# Autodesk Inventor assembly: Main Body
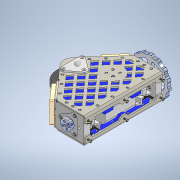
[picture p0: Inventor's stored thumbnail of the model, 180x180]
Saved by Autodesk Inventor 2022 (Build 260153000, 153)
## iProperties
Created: 2022-08-09
Part Number: Main Body
Document SubType Name: Assembly
Designer: Nick
Mass: 1334.27 g
Surface Area: 2820.47 cm^2
Volume: 520.306 cm^3
Density: 2.56439 g/cm^3
Author: Nick
## Documents named in this file (31)
- Y:\Projects\BattleBot\Main Body.iam
- Y:\Projects\BattleBot\Battery.ipt
- Y:\Projects\BattleBot\ESC.ipt
- Y:\Projects\BattleBot\Motor.ipt
- Y:\Projects\BattleBot\RC Reciever.ipt
- Y:\Projects\BattleBot\Base Plate.ipt
- Y:\Projects\BattleBot\Weapon.ipt
- Y:\Projects\BattleBot\Brushless Motor.ipt
- Y:\Projects\BattleBot\Brushed ESC.ipt
- Y:\Projects\BattleBot\Bottom Substructure.ipt
- Y:\Projects\BattleBot\Wheel.ipt
- Y:\Projects\BattleBot\6901 Bearing.ipt
- Y:\Projects\BattleBot\GT2 Pulley 16T.ipt
- Y:\Projects\BattleBot\Motor Mount Insert.ipt
- Y:\Projects\BattleBot\Mount Side.ipt
- Y:\Projects\BattleBot\Top Stubstructure.ipt
- Y:\Projects\BattleBot\Shaft.ipt
- Y:\Projects\BattleBot\Key.ipt
- Y:\Projects\BattleBot\ESC Mount.ipt
- Y:\Projects\BattleBot\Shaft Collar.ipt
- Y:\Projects\BattleBot\Wheel Hub.ipt
- Y:\Projects\BattleBot\Front Armor.ipt
- Y:\Projects\BattleBot\Rear Armor.ipt
- Y:\Projects\BattleBot\M3 Heat Set Insert.ipt
- Y:\Projects\BattleBot\M3 x 8 mm FHCS.ipt
- Y:\Projects\Mini_Sand_Table\Hardware\M3\Bolts\M3 x 8 mm FHCS.ipt
- Y:\Projects\BattleBot\M3 x 12 mm FHCS.ipt
- Y:\Projects\BattleBot\Motor Clamp.ipt
- Y:\Projects\BattleBot\Pulley.ipt
- Y:\Projects\BattleBot\Idle Ball Mount.ipt
- Y:\Projects\BattleBot\Ball.ipt
## Components (183 placed, 29 different names)
1. Battery:1 — Mate:146, Mate:182, Mate:189, Flush:39
2. ESC:1 — Mate:168, Mate:189, Flush:39, Mate:191
3. Base Plate:1 — Mate:42, Mate:95, Insert:15, Mate:104, Mate:105, Mate:139, Flush:28, Mate:140, Flush:29, Insert:123, Insert:124, Insert:125, Insert:126, Insert:127, Insert:128, Insert:129, Insert:130, Insert:131, Insert:132, Insert:133, Insert:134, Insert:135, Insert:136, Insert:137, Insert:138, Insert:183, Insert:184, Insert:185, Insert:189, Insert:190
4. Weapon:1 — Mate:145, Mate:159, Insert:33, Angle:1, Mate:187
5. Brushless Motor:1 — Insert:26, Insert:32
6. Motor:2 — Insert:22, Insert:36, Angle:2
7. Motor:3 — Insert:21, Insert:39, Angle:3
8. Brushed ESC:1 — Mate:128, Mate:132, Flush:37
9. Brushed ESC:2 — Mate:150, Mate:161
10. Bottom Substructure:2 — Mate:42, Mate:95, Mate:128, Mate:144, Flush:32, Mate:146, Mate:161, Mate:162, Mate:165, Mate:182, Insert:42, Insert:43, Insert:44, Insert:45, Insert:46, Insert:47, Insert:48, Insert:51, Insert:52, Insert:53, Insert:56, Insert:57, Insert:99, Insert:100, Insert:105, Insert:106, Mate:190
11. Base Plate:2 — Mate:125, Insert:32, Mate:173, Mate:174, Mate:178, Mate:179, Insert:107, Insert:108, Insert:109, Insert:110, Insert:111, Insert:112, Insert:113, Insert:114, Insert:115, Insert:116, Insert:117, Insert:118, Insert:119, Insert:120, Insert:121, Insert:122, Insert:139, Insert:140, Insert:141, Insert:142, Mate:183, Mate:185, Insert:186, Insert:187, Insert:188, Insert:192, Insert:193
12. Wheel:1 — Insert:34, Insert:195
13. Wheel:2 — Insert:37
14. 6901 Bearing:1 — Insert:15, Insert:27
15. GT2 Pulley 16T:1 — Insert:26
16. Motor Mount Insert:1 — Insert:22, Insert:30, Insert:31, Insert:147, Insert:148, Insert:149
17. Mount Side:1 — Mate:104, Mate:140, Flush:29, Mate:144, Mate:150, Mate:164, Mate:166, Insert:30, Insert:31, Flush:38, Insert:86, Insert:87, Insert:88, Insert:89, Insert:90, Insert:91, Insert:92, Insert:93, Insert:94, Insert:95, Insert:96, Insert:98
18. Mount Side:2 — Mate:105, Mate:132, Mate:139, Flush:28, Flush:30, Mate:141, Mate:163, Flush:36, Insert:28, Insert:29, Mate:180, Insert:72, Insert:73, Insert:74, Insert:75, Insert:76, Insert:77, Insert:78, Insert:79, Insert:81, Insert:82, Insert:83, Insert:84
19. Motor Mount Insert:3 — Insert:21, Insert:28, Insert:29, Insert:150, Insert:151, Insert:152
20. 6901 Bearing:2 — Insert:25
21. Top Stubstructure:1 — Mate:125, Insert:25, Flush:30, Mate:141, Insert:58, Insert:59, Insert:60, Insert:61, Insert:62, Insert:63, Insert:64, Insert:65, Insert:66, Insert:67, Insert:68, Insert:69, Insert:70, Insert:71, Insert:101, Insert:102, Insert:103, Insert:104
22. Shaft:1 — Insert:27, Mate:157, Mate:158, Mate:159, Mate:186
23. Key:1 — Mate:157, Mate:158, Angle:1, Angle:4
24. ESC Mount:1 — Mate:162, Mate:163, Flush:36, Flush:37, Insert:173, Insert:174, Insert:180, Angle:3
25. ESC Mount:2 — Mate:164, Mate:165, Mate:166, Mate:168, Insert:171, Insert:172, Insert:175, Insert:176, Angle:2
26. Shaft Collar:1 — Insert:33
27. Wheel Hub:1 — Insert:34, Insert:36, Insert:195
28. Wheel Hub:2 — Insert:37, Insert:39
29. Front Armor:1 — Mate:173, Flush:38, Mate:174, Mate:184, Insert:163, Insert:164, Insert:165, Insert:166
30. Front Armor:2 — Mate:183, Mate:184, Mate:185, Insert:167, Insert:168, Insert:169, Insert:170
31. Rear Armor:1 — Mate:178, Mate:179, Mate:180
32. Motor Clamp:1 — Insert:175, Insert:176, Insert:177, Insert:178
33. Motor Clamp:2 — Insert:179, Insert:180, Insert:181, Insert:182
34. Pulley:1 — Mate:186, Angle:4, Mate:187
35. Idle Ball Mount:1 — Insert:189, Insert:190, Insert:191
36. Idle Ball Mount:2 — Insert:192, Insert:193, Insert:194
37. Ball:1 — Insert:191
38. Ball:2 — Insert:194
39. RC Reciever:1 — Mate:190, Mate:191
40. M3 Heat Set Insert:67 — Insert:171
41. M3 Heat Set Insert:68 — Insert:172
42. M3 Heat Set Insert:69 — Insert:174
43. M3 Heat Set Insert:70 — Insert:173, Insert:179
44. M3 Heat Set Insert:1 — Insert:48
45. M3 Heat Set Insert:2 — Insert:47
46. M3 Heat Set Insert:3 — Insert:46
47. M3 Heat Set Insert:4 — Insert:45
48. M3 Heat Set Insert:5
49. M3 Heat Set Insert:6 — Insert:42
50. M3 Heat Set Insert:7 — Insert:43
51. M3 Heat Set Insert:8 — Insert:44
52. M3 Heat Set Insert:9
53. M3 Heat Set Insert:10 — Insert:51
54. M3 Heat Set Insert:11 — Insert:52
55. M3 Heat Set Insert:12 — Insert:53
56. M3 Heat Set Insert:13 — Insert:56
57. M3 Heat Set Insert:14
58. M3 Heat Set Insert:15
59. M3 Heat Set Insert:16
60. M3 Heat Set Insert:17
61. M3 Heat Set Insert:18 — Insert:57
62. M3 Heat Set Insert:19 — Insert:58
63. M3 Heat Set Insert:20 — Insert:59
64. M3 Heat Set Insert:21 — Insert:60
65. M3 Heat Set Insert:22 — Insert:61
66. M3 Heat Set Insert:23 — Insert:67
67. M3 Heat Set Insert:24 — Insert:66
68. M3 Heat Set Insert:25 — Insert:65
69. M3 Heat Set Insert:26 — Insert:64
70. M3 Heat Set Insert:27 — Insert:68
71. M3 Heat Set Insert:28 — Insert:69
72. M3 Heat Set Insert:29 — Insert:70
73. M3 Heat Set Insert:30 — Insert:71
74. M3 Heat Set Insert:31 — Insert:63
75. M3 Heat Set Insert:32 — Insert:62
76. M3 Heat Set Insert:33 — Insert:77
77. M3 Heat Set Insert:34 — Insert:76
78. M3 Heat Set Insert:35 — Insert:75
79. M3 Heat Set Insert:36 — Insert:78
80. M3 Heat Set Insert:37 — Insert:73
81. M3 Heat Set Insert:38 — Insert:72
82. M3 Heat Set Insert:39 — Insert:79
83. M3 Heat Set Insert:40 — Insert:74
84. M3 Heat Set Insert:41
85. M3 Heat Set Insert:42 — Insert:82
86. M3 Heat Set Insert:43 — Insert:83
87. M3 Heat Set Insert:44 — Insert:81
88. M3 Heat Set Insert:45 — Insert:84
89. M3 Heat Set Insert:46 — Insert:92
90. M3 Heat Set Insert:47 — Insert:87
91. M3 Heat Set Insert:48 — Insert:86
92. M3 Heat Set Insert:49 — Insert:98
93. M3 Heat Set Insert:50 — Insert:95
94. M3 Heat Set Insert:51 — Insert:91
95. M3 Heat Set Insert:52 — Insert:96
96. M3 Heat Set Insert:53 — Insert:94
97. M3 Heat Set Insert:54 — Insert:88
98. M3 Heat Set Insert:55 — Insert:90
99. M3 Heat Set Insert:56 — Insert:89
100. M3 Heat Set Insert:57 — Insert:93
101. M3 Heat Set Insert:58
102. M3 Heat Set Insert:59 — Insert:99
103. M3 Heat Set Insert:60 — Insert:100
104. M3 Heat Set Insert:61 — Insert:102
105. M3 Heat Set Insert:62 — Insert:101
106. M3 Heat Set Insert:63 — Insert:103
107. M3 Heat Set Insert:64 — Insert:105
108. M3 Heat Set Insert:65 — Insert:104
109. M3 Heat Set Insert:66 — Insert:106
110. M3 x 8 mm FHCS:51 — Insert:183
111. M3 x 8 mm FHCS:52 — Insert:184
112. M3 x 8 mm FHCS:53 — Insert:185
113. M3 x 8 mm FHCS:54 — Insert:186
114. M3 x 8 mm FHCS:55 — Insert:188
115. M3 x 8 mm FHCS:56 — Insert:187
116. M3 x 8 mm FHCS:1 — Insert:107
117. M3 x 8 mm FHCS:2 — Insert:108
118. M3 x 8 mm FHCS:3 — Insert:110
119. M3 x 8 mm FHCS:4 — Insert:109
120. M3 x 8 mm FHCS:5 — Insert:111
121. M3 x 8 mm FHCS:6 — Insert:112
122. M3 x 8 mm FHCS:7 — Insert:113
123. M3 x 8 mm FHCS:8 — Insert:114
124. M3 x 8 mm FHCS:9 — Insert:115
125. M3 x 8 mm FHCS:10 — Insert:116
126. M3 x 8 mm FHCS:11 — Insert:118
127. M3 x 8 mm FHCS:12 — Insert:119
128. M3 x 8 mm FHCS:13 — Insert:117
129. M3 x 8 mm FHCS:14 — Insert:120
130. M3 x 8 mm FHCS:15 — Insert:123
131. M3 x 8 mm FHCS:16 — Insert:122
132. M3 x 8 mm FHCS:17 — Insert:121
133. M3 x 8 mm FHCS:18 — Insert:124
134. M3 x 8 mm FHCS:19 — Insert:125
135. M3 x 8 mm FHCS:20 — Insert:126
136. M3 x 8 mm FHCS:21 — Insert:127
137. M3 x 8 mm FHCS:22 — Insert:128
138. M3 x 8 mm FHCS:23 — Insert:129
139. M3 x 8 mm FHCS:24 — Insert:130
140. M3 x 8 mm FHCS:25 — Insert:131
141. M3 x 8 mm FHCS:26 — Insert:132
142. M3 x 8 mm FHCS:27 — Insert:133
143. M3 x 8 mm FHCS:28 — Insert:134
144. M3 x 8 mm FHCS:29 — Insert:138
145. M3 x 8 mm FHCS:30 — Insert:137
146. M3 x 8 mm FHCS:31 — Insert:136
147. M3 x 8 mm FHCS:32 — Insert:135
148. M3 x 8 mm FHCS:33 — Insert:139
149. M3 x 8 mm FHCS:34 — Insert:140
150. M3 x 8 mm FHCS:35 — Insert:142
151. M3 x 8 mm FHCS:36 — Insert:141
152. M3 x 8 mm FHCS:37 — Insert:147
153. M3 x 8 mm FHCS:38 — Insert:148
154. M3 x 8 mm FHCS:39
155. M3 x 8 mm FHCS:40 — Insert:149
156. M3 x 8 mm FHCS:41
157. M3 x 8 mm FHCS:42
158. M3 x 8 mm FHCS:43
159. M3 x 8 mm FHCS:44
160. M3 x 8 mm FHCS:45 — Insert:152
161. M3 x 8 mm FHCS:46
162. M3 x 8 mm FHCS:47
163. M3 x 8 mm FHCS:48 — Insert:150
164. M3 x 8 mm FHCS:49 — Insert:151
165. M3 x 8 mm FHCS:50
166. M3 x 12 mm FHCS:15 — Insert:177
167. M3 x 12 mm FHCS:16 — Insert:178
168. M3 x 12 mm FHCS:17 — Insert:182
169. M3 x 12 mm FHCS:18 — Insert:181
170. M3 x 12 mm FHCS:1
171. M3 x 12 mm FHCS:2
172. M3 x 12 mm FHCS:3
173. M3 x 12 mm FHCS:4
174. M3 x 12 mm FHCS:5
175. M3 x 12 mm FHCS:6
176. M3 x 12 mm FHCS:7 — Insert:168
177. M3 x 12 mm FHCS:8 — Insert:167
178. M3 x 12 mm FHCS:9 — Insert:169
179. M3 x 12 mm FHCS:10 — Insert:170
180. M3 x 12 mm FHCS:11 — Insert:164
181. M3 x 12 mm FHCS:12 — Insert:163
182. M3 x 12 mm FHCS:13 — Insert:165
183. M3 x 12 mm FHCS:14 — Insert:166
## Relationships (199: Insert 149, Mate 38, Flush 8, Angle 4)
- Mate:42: Base Plate:1 ↔ Bottom Substructure:2
- Mate:95: Base Plate:1 ↔ Bottom Substructure:2
- Insert:15: Base Plate:1 ↔ 6901 Bearing:1
- Mate:104: Base Plate:1 ↔ Mount Side:1
- Mate:105: Base Plate:1 ↔ Mount Side:2
- Insert:21: Motor:3 ↔ Motor Mount Insert:3
- Insert:22: Motor:2 ↔ Motor Mount Insert:1
- Mate:125: Base Plate:2 ↔ Top Stubstructure:1
- Insert:25: 6901 Bearing:2 ↔ Top Stubstructure:1
- Mate:128: Brushed ESC:1 ↔ Bottom Substructure:2
- Mate:132: Brushed ESC:1 ↔ Mount Side:2
- Mate:139: Base Plate:1 ↔ Mount Side:2
- Flush:28: Base Plate:1 ↔ Mount Side:2
- Mate:140: Base Plate:1 ↔ Mount Side:1
- Flush:29: Base Plate:1 ↔ Mount Side:1
- Flush:30: Mount Side:2 ↔ Top Stubstructure:1
- Mate:141: Mount Side:2 ↔ Top Stubstructure:1
- Mate:144: Bottom Substructure:2 ↔ Mount Side:1
- Flush:32 (15.5 mm): Bottom Substructure:2
- Mate:145: Weapon:1
- Mate:146: Battery:1 ↔ Bottom Substructure:2
- Mate:150: Brushed ESC:2 ↔ Mount Side:1
- Insert:26: Brushless Motor:1 ↔ GT2 Pulley 16T:1
- Insert:27: 6901 Bearing:1 ↔ Shaft:1
- Mate:157: Shaft:1 ↔ Key:1
- Mate:158: Shaft:1 ↔ Key:1
- Mate:159: Weapon:1 ↔ Shaft:1
- Mate:161: Brushed ESC:2 ↔ Bottom Substructure:2
- Mate:162: Bottom Substructure:2 ↔ ESC Mount:1
- Mate:163: Mount Side:2 ↔ ESC Mount:1
- Flush:36: Mount Side:2 ↔ ESC Mount:1
- Flush:37: Brushed ESC:1 ↔ ESC Mount:1
- Mate:164: Mount Side:1 ↔ ESC Mount:2
- Mate:165: Bottom Substructure:2 ↔ ESC Mount:2
- Mate:166: Mount Side:1 ↔ ESC Mount:2
- Mate:168 (1 mm): ESC:1 ↔ ESC Mount:2
- Insert:28: Mount Side:2 ↔ Motor Mount Insert:3
- Insert:29: Mount Side:2 ↔ Motor Mount Insert:3
- Insert:30: Motor Mount Insert:1 ↔ Mount Side:1
- Insert:31: Motor Mount Insert:1 ↔ Mount Side:1
- Insert:32: Brushless Motor:1 ↔ Base Plate:2
- Insert:33: Weapon:1 ↔ Shaft Collar:1
- Angle:1 (180 deg): Weapon:1 ↔ Key:1
- Insert:34: Wheel:1 ↔ Wheel Hub:1
- Insert:36: Motor:2 ↔ Wheel Hub:1
- Insert:37: Wheel:2 ↔ Wheel Hub:2
- Insert:39: Motor:3 ↔ Wheel Hub:2
- Mate:173: Base Plate:2 ↔ Front Armor:1
- Flush:38: Mount Side:1 ↔ Front Armor:1
- Mate:174: Base Plate:2 ↔ Front Armor:1
- Mate:178: Base Plate:2 ↔ Rear Armor:1
- Mate:179: Base Plate:2 ↔ Rear Armor:1
- Mate:180: Mount Side:2 ↔ Rear Armor:1
- Mate:182: Battery:1 ↔ Bottom Substructure:2
- Insert:42: Bottom Substructure:2 ↔ M3 Heat Set Insert:6
- Insert:43: Bottom Substructure:2 ↔ M3 Heat Set Insert:7
- Insert:44: Bottom Substructure:2 ↔ M3 Heat Set Insert:8
- Insert:45: Bottom Substructure:2 ↔ M3 Heat Set Insert:4
- Insert:46: Bottom Substructure:2 ↔ M3 Heat Set Insert:3
- Insert:47: Bottom Substructure:2 ↔ M3 Heat Set Insert:2
- Insert:48: Bottom Substructure:2 ↔ M3 Heat Set Insert:1
- Insert:51: Bottom Substructure:2 ↔ M3 Heat Set Insert:10
- Insert:52: Bottom Substructure:2 ↔ M3 Heat Set Insert:11
- Insert:53: Bottom Substructure:2 ↔ M3 Heat Set Insert:12
- Insert:56: Bottom Substructure:2 ↔ M3 Heat Set Insert:13
- Insert:57: Bottom Substructure:2 ↔ M3 Heat Set Insert:18
- Insert:58: Top Stubstructure:1 ↔ M3 Heat Set Insert:19
- Insert:59: Top Stubstructure:1 ↔ M3 Heat Set Insert:20
- Insert:60: Top Stubstructure:1 ↔ M3 Heat Set Insert:21
- Insert:61: Top Stubstructure:1 ↔ M3 Heat Set Insert:22
- Insert:62: Top Stubstructure:1 ↔ M3 Heat Set Insert:32
- Insert:63: Top Stubstructure:1 ↔ M3 Heat Set Insert:31
- Insert:64: Top Stubstructure:1 ↔ M3 Heat Set Insert:26
- Insert:65: Top Stubstructure:1 ↔ M3 Heat Set Insert:25
- Insert:66: Top Stubstructure:1 ↔ M3 Heat Set Insert:24
- Insert:67: Top Stubstructure:1 ↔ M3 Heat Set Insert:23
- Insert:68: Top Stubstructure:1 ↔ M3 Heat Set Insert:27
- Insert:69: Top Stubstructure:1 ↔ M3 Heat Set Insert:28
- Insert:70: Top Stubstructure:1 ↔ M3 Heat Set Insert:29
- Insert:71: Top Stubstructure:1 ↔ M3 Heat Set Insert:30
- Insert:72: Mount Side:2 ↔ M3 Heat Set Insert:38
- Insert:73: Mount Side:2 ↔ M3 Heat Set Insert:37
- Insert:74: Mount Side:2 ↔ M3 Heat Set Insert:40
- Insert:75: Mount Side:2 ↔ M3 Heat Set Insert:35
- Insert:76: Mount Side:2 ↔ M3 Heat Set Insert:34
- Insert:77: Mount Side:2 ↔ M3 Heat Set Insert:33
- Insert:78: Mount Side:2 ↔ M3 Heat Set Insert:36
- Insert:79: Mount Side:2 ↔ M3 Heat Set Insert:39
- Insert:81: Mount Side:2 ↔ M3 Heat Set Insert:44
- Insert:82: Mount Side:2 ↔ M3 Heat Set Insert:42
- Insert:83: Mount Side:2 ↔ M3 Heat Set Insert:43
- Insert:84: Mount Side:2 ↔ M3 Heat Set Insert:45
- Insert:86: Mount Side:1 ↔ M3 Heat Set Insert:48
- Insert:87: Mount Side:1 ↔ M3 Heat Set Insert:47
- Insert:88: Mount Side:1 ↔ M3 Heat Set Insert:54
- Insert:89: Mount Side:1 ↔ M3 Heat Set Insert:56
- Insert:90: Mount Side:1 ↔ M3 Heat Set Insert:55
- Insert:91: Mount Side:1 ↔ M3 Heat Set Insert:51
- Insert:92: Mount Side:1 ↔ M3 Heat Set Insert:46
- Insert:93: Mount Side:1 ↔ M3 Heat Set Insert:57
- Insert:94: Mount Side:1 ↔ M3 Heat Set Insert:53
- Insert:95: Mount Side:1 ↔ M3 Heat Set Insert:50
- Insert:96: Mount Side:1 ↔ M3 Heat Set Insert:52
- Insert:98: Mount Side:1 ↔ M3 Heat Set Insert:49
- Insert:99: Bottom Substructure:2 ↔ M3 Heat Set Insert:59
- Insert:100: Bottom Substructure:2 ↔ M3 Heat Set Insert:60
- Insert:101: Top Stubstructure:1 ↔ M3 Heat Set Insert:62
- Insert:102: Top Stubstructure:1 ↔ M3 Heat Set Insert:61
- Insert:103: Top Stubstructure:1 ↔ M3 Heat Set Insert:63
- Insert:104: Top Stubstructure:1 ↔ M3 Heat Set Insert:65
- Insert:105: Bottom Substructure:2 ↔ M3 Heat Set Insert:64
- Insert:106: Bottom Substructure:2 ↔ M3 Heat Set Insert:66
- Insert:107: Base Plate:2 ↔ M3 x 8 mm FHCS:1
- Insert:108: Base Plate:2 ↔ M3 x 8 mm FHCS:2
- Insert:109: Base Plate:2 ↔ M3 x 8 mm FHCS:4
- Insert:110: Base Plate:2 ↔ M3 x 8 mm FHCS:3
- Insert:111: Base Plate:2 ↔ M3 x 8 mm FHCS:5
- Insert:112: Base Plate:2 ↔ M3 x 8 mm FHCS:6
- Insert:113: Base Plate:2 ↔ M3 x 8 mm FHCS:7
- Insert:114: Base Plate:2 ↔ M3 x 8 mm FHCS:8
- Insert:115: Base Plate:2 ↔ M3 x 8 mm FHCS:9
- Insert:116: Base Plate:2 ↔ M3 x 8 mm FHCS:10
- Insert:117: Base Plate:2 ↔ M3 x 8 mm FHCS:13
- Insert:118: Base Plate:2 ↔ M3 x 8 mm FHCS:11
- Insert:119: Base Plate:2 ↔ M3 x 8 mm FHCS:12
- Insert:120: Base Plate:2 ↔ M3 x 8 mm FHCS:14
- Insert:121: Base Plate:2 ↔ M3 x 8 mm FHCS:17
- Insert:122: Base Plate:2 ↔ M3 x 8 mm FHCS:16
- Insert:123: Base Plate:1 ↔ M3 x 8 mm FHCS:15
- Insert:124: Base Plate:1 ↔ M3 x 8 mm FHCS:18
- Insert:125: Base Plate:1 ↔ M3 x 8 mm FHCS:19
- Insert:126: Base Plate:1 ↔ M3 x 8 mm FHCS:20
- Insert:127: Base Plate:1 ↔ M3 x 8 mm FHCS:21
- Insert:128: Base Plate:1 ↔ M3 x 8 mm FHCS:22
- Insert:129: Base Plate:1 ↔ M3 x 8 mm FHCS:23
- Insert:130: Base Plate:1 ↔ M3 x 8 mm FHCS:24
- Insert:131: Base Plate:1 ↔ M3 x 8 mm FHCS:25
- Insert:132: Base Plate:1 ↔ M3 x 8 mm FHCS:26
- Insert:133: Base Plate:1 ↔ M3 x 8 mm FHCS:27
- Insert:134: Base Plate:1 ↔ M3 x 8 mm FHCS:28
- Insert:135: Base Plate:1 ↔ M3 x 8 mm FHCS:32
- Insert:136: Base Plate:1 ↔ M3 x 8 mm FHCS:31
- Insert:137: Base Plate:1 ↔ M3 x 8 mm FHCS:30
- Insert:138: Base Plate:1 ↔ M3 x 8 mm FHCS:29
- Insert:139: Base Plate:2 ↔ M3 x 8 mm FHCS:33
- Insert:140: Base Plate:2 ↔ M3 x 8 mm FHCS:34
- Insert:141: Base Plate:2 ↔ M3 x 8 mm FHCS:36
- Insert:142: Base Plate:2 ↔ M3 x 8 mm FHCS:35
- Insert:147: Motor Mount Insert:1 ↔ M3 x 8 mm FHCS:37
- Insert:148: Motor Mount Insert:1 ↔ M3 x 8 mm FHCS:38
- Insert:149: Motor Mount Insert:1 ↔ M3 x 8 mm FHCS:40
- Insert:150: Motor Mount Insert:3 ↔ M3 x 8 mm FHCS:48
- Insert:151: Motor Mount Insert:3 ↔ M3 x 8 mm FHCS:49
- Insert:152: Motor Mount Insert:3 ↔ M3 x 8 mm FHCS:45
- Mate:183: Base Plate:2 ↔ Front Armor:2
- Mate:184: Front Armor:1 ↔ Front Armor:2
- Mate:185: Base Plate:2 ↔ Front Armor:2
- Insert:163: Front Armor:1 ↔ M3 x 12 mm FHCS:12
- Insert:164: Front Armor:1 ↔ M3 x 12 mm FHCS:11
- Insert:165: Front Armor:1 ↔ M3 x 12 mm FHCS:13
- Insert:166: Front Armor:1 ↔ M3 x 12 mm FHCS:14
- Insert:167: Front Armor:2 ↔ M3 x 12 mm FHCS:8
- Insert:168: Front Armor:2 ↔ M3 x 12 mm FHCS:7
- Insert:169: Front Armor:2 ↔ M3 x 12 mm FHCS:9
- Insert:170: Front Armor:2 ↔ M3 x 12 mm FHCS:10
- Insert:171: ESC Mount:2 ↔ M3 Heat Set Insert:67
- Insert:172: ESC Mount:2 ↔ M3 Heat Set Insert:68
- Insert:173: ESC Mount:1 ↔ M3 Heat Set Insert:70
- Insert:174: ESC Mount:1 ↔ M3 Heat Set Insert:69
- Insert:175: ESC Mount:2 ↔ Motor Clamp:1
- Insert:176: ESC Mount:2 ↔ Motor Clamp:1
- Insert:177: Motor Clamp:1 ↔ M3 x 12 mm FHCS:15
- Insert:178: Motor Clamp:1 ↔ M3 x 12 mm FHCS:16
- Insert:179: Motor Clamp:2 ↔ M3 Heat Set Insert:70
- Insert:180: ESC Mount:1 ↔ Motor Clamp:2
- Insert:181: Motor Clamp:2 ↔ M3 x 12 mm FHCS:18
- Insert:182: Motor Clamp:2 ↔ M3 x 12 mm FHCS:17
- Angle:2 (0 deg): Motor:2 ↔ ESC Mount:2
- Angle:3 (0 deg): Motor:3 ↔ ESC Mount:1
- Mate:186: Shaft:1 ↔ Pulley:1
- Angle:4 (180 deg): Key:1 ↔ Pulley:1
- Mate:187: Weapon:1 ↔ Pulley:1
- Insert:183: Base Plate:1 ↔ M3 x 8 mm FHCS:51
- Insert:184: Base Plate:1 ↔ M3 x 8 mm FHCS:52
- Insert:185: Base Plate:1 ↔ M3 x 8 mm FHCS:53
- Insert:186: Base Plate:2 ↔ M3 x 8 mm FHCS:54
- Insert:187: Base Plate:2 ↔ M3 x 8 mm FHCS:56
- Insert:188: Base Plate:2 ↔ M3 x 8 mm FHCS:55
- Insert:189: Base Plate:1 ↔ Idle Ball Mount:1
- Insert:190: Base Plate:1 ↔ Idle Ball Mount:1
- Insert:191: Idle Ball Mount:1 ↔ Ball:1
- Mate:189: Battery:1 ↔ ESC:1
- Flush:39: Battery:1 ↔ ESC:1
- Insert:192: Base Plate:2 ↔ Idle Ball Mount:2
- Insert:193: Base Plate:2 ↔ Idle Ball Mount:2
- Insert:194: Idle Ball Mount:2 ↔ Ball:2
- Mate:190: Bottom Substructure:2 ↔ RC Reciever:1
- Mate:191: ESC:1 ↔ RC Reciever:1
- Insert:195: Wheel:1 ↔ Wheel Hub:1
